# Autodesk Inventor assembly: NEO550.ver1-1111-2020
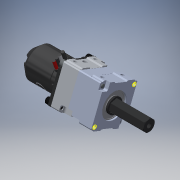
[picture p0: Inventor's stored thumbnail of the model, 180x180]
Saved by Autodesk Inventor 2018 (Build 220112000, 112)
## iProperties
Created: 2020-01-14
Part Number: NEO550.ver1-1111-2020
Document SubType Name: Assembly
Designer: Power Hawks CADD
Author: Power Hawks CADD
## Documents named in this file (3)
- E:\GrabCAD\Power Hawks CAD\2020 Infinite Recharge\Intake\Parts\NEO550.ver1-1111-2020.iam
- E:\GrabCAD\Power Hawks CAD\2020 Infinite Recharge\Intake\Parts\REV-21-1651.ipt
- E:\GrabCAD\Power Hawks CAD\Resources\VEXpro Resources\Motors\Versaplanetary Gearbox with 775 Pro\v2-VersaPlanetary-3in-1stage-with-775pro-20161031.iam
## Components (2 placed, 2 different names)
1. REV-21-1651:1 — Cylindrical:1, Mate:1
2. v2-VersaPlanetary-3in-1stage-with-775pro-20161031:1 [sub-assembly] — Cylindrical:1, Mate:1
## Relationships (2: CylindricalJoint 1, Mate 1)
- Cylindrical:1: REV-21-1651:1 ↔ v2-VersaPlanetary-3in-1stage-with-775pro-20161031:1
- Mate:1: REV-21-1651:1 ↔ v2-VersaPlanetary-3in-1stage-with-775pro-20161031:1
